# Autodesk Inventor assembly: Caja_Reductora
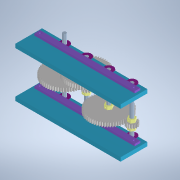
[picture p0: Inventor's stored thumbnail of the model, 180x180]
Saved by Autodesk Inventor 2022 (Build 260153000, 153)
## iProperties
Created: 2022-02-21
Part Number: Caja_Reductora
Document SubType Name: Assembly
Designer: katha
Author: katha
## Documents named in this file (11)
- C:\Users\katha\OneDrive\Escritorio\Mini_Proyecto_Diseno\Diseno_18012\Modelo_MPD\Caja_Reductora.iam
- C:\Users\katha\OneDrive\Escritorio\Mini_Proyecto_Diseno\Diseno_18012\Modelo_MPD\Engranajes_1_4.ipt
- C:\Users\katha\OneDrive\Escritorio\Mini_Proyecto_Diseno\Diseno_18012\Modelo_MPD\Engranajes_1_5.ipt
- C:\Users\katha\OneDrive\Escritorio\Mini_Proyecto_Diseno\Diseno_18012\Modelo_MPD\Eje1.ipt
- C:\Users\katha\OneDrive\Escritorio\Mini_Proyecto_Diseno\Diseno_18012\Modelo_MPD\Eje2.ipt
- C:\Users\katha\OneDrive\Escritorio\Mini_Proyecto_Diseno\Diseno_18012\Modelo_MPD\Hombro_Ejes.ipt
- C:\Users\katha\OneDrive\Escritorio\Mini_Proyecto_Diseno\Diseno_18012\Modelo_MPD\Rodamiento_Ejes.ipt
- C:\Users\katha\OneDrive\Escritorio\Mini_Proyecto_Diseno\Diseno_18012\Modelo_MPD\Carcasa_CajaR_Lateral1.ipt
- C:\Users\katha\OneDrive\Escritorio\Mini_Proyecto_Diseno\Diseno_18012\Modelo_MPD\Eje_Entrada.ipt
- C:\Users\katha\OneDrive\Escritorio\Mini_Proyecto_Diseno\Diseno_18012\Modelo_MPD\Eje_Salida.ipt
- C:\Users\katha\OneDrive\Escritorio\Mini_Proyecto_Diseno\Diseno_18012\Modelo_MPD\Carcasa_Tope.ipt
## Components (33 placed, 10 different names)
1. Engranajes_1_4:1 — Mate:2, Mate:3, Mate:35, Mate:36, Mate:43, Mate:44, Mate:63, Mate:64
2. Engranajes_1_5:1 — Mate:8, Mate:9, Mate:41, Mate:42, Mate:45, Mate:46, Mate:70, Mate:71
3. Engranajes_1_5:2 — Mate:1, Mate:4, Mate:5, Mate:6, Mate:7, Mate:37, Mate:38, Mate:39, Mate:40
4. Eje1:1 — Mate:1, Mate:2, Mate:3, Mate:4, Mate:5, Mate:10, Mate:11, Mate:12, Mate:13, Mate:14, Mate:15, Mate:16, Mate:17, Flush:1, Flush:2, Mate:27, Mate:28, Flush:4, Mate:31, Mate:32, Flush:6, Flush:7, Flush:10, Flush:11
5. Eje2:1 — Mate:6, Mate:7, Mate:8, Mate:9, Mate:18, Mate:19, Mate:20, Mate:21, Mate:22, Mate:23, Mate:24, Mate:25, Mate:26, Flush:1, Flush:3, Mate:29, Mate:30, Flush:5, Mate:33, Mate:34, Flush:8, Flush:9, Flush:11, Flush:12
6. Hombro_Ejes:1 — Mate:10, Mate:11, Flush:7, Mate:37
7. Hombro_Ejes:2 — Mate:12, Mate:13, Mate:38
8. Hombro_Ejes:3 — Mate:14, Mate:15, Mate:36
9. Hombro_Ejes:4 — Mate:16, Mate:17, Flush:6, Mate:35
10. Hombro_Ejes:5 — Mate:22, Mate:25, Mate:26, Mate:40
11. Hombro_Ejes:6 — Mate:23, Mate:24, Mate:39
12. Hombro_Ejes:7 — Mate:18, Mate:19, Flush:8, Mate:41
13. Hombro_Ejes:8 — Mate:20, Mate:21, Mate:42
14. Rodamiento_Ejes:1 — Flush:3, Mate:29, Mate:30, Flush:16
15. Rodamiento_Ejes:2 — Flush:2, Mate:27, Mate:28
16. Rodamiento_Ejes:3 — Flush:5, Mate:33, Mate:34
17. Rodamiento_Ejes:4 — Flush:4, Mate:31, Mate:32, Flush:13, Flush:19
18. Carcasa_CajaR_Lateral1:1 — Flush:9, Flush:17, Flush:18, Flush:20, Mate:56
19. Eje_Entrada:1 — Mate:43, Mate:44, Flush:10, Mate:47, Mate:48, Mate:52, Mate:53, Flush:15, Mate:59, Mate:60, Mate:61, Mate:62
20. Eje_Salida:1 — Mate:45, Mate:46, Flush:12, Mate:49, Mate:50, Mate:51, Flush:14, Mate:54, Mate:55, Mate:65, Mate:66, Mate:67, Mate:68, Mate:69
21. Rodamiento_Ejes:5 — Mate:47, Mate:48, Flush:13
22. Rodamiento_Ejes:6 — Mate:49, Mate:50, Mate:51, Flush:14
23. Rodamiento_Ejes:7 — Mate:52, Mate:53, Flush:15
24. Rodamiento_Ejes:8 — Mate:54, Mate:55, Flush:16
25. Carcasa_CajaR_Lateral1:2 — Flush:17, Flush:18, Flush:19, Mate:57, Mate:58
26. Carcasa_Tope:1 — Flush:20, Flush:21, Flush:22, Flush:23, Flush:24, Flush:25
27. Carcasa_Tope:2 — Flush:21, Flush:22, Mate:56
28. Carcasa_Tope:3 — Flush:23, Flush:24, Flush:26, Mate:57
29. Carcasa_Tope:4 — Flush:25, Flush:26, Mate:58
30. Hombro_Ejes:9 — Mate:59, Mate:60, Mate:64
31. Hombro_Ejes:10 — Mate:61, Mate:62, Mate:63
32. Hombro_Ejes:11 — Mate:65, Mate:68, Mate:69, Mate:70
33. Hombro_Ejes:12 — Mate:66, Mate:67, Mate:71
## Relationships (97: Mate 71, Flush 26)
- Mate:1 (0.3 mm): Engranajes_1_5:2 ↔ Eje1:1
- Mate:2 (0.3 mm): Engranajes_1_4:1 ↔ Eje1:1
- Mate:3 (0.3 mm): Engranajes_1_4:1 ↔ Eje1:1
- Mate:4 (0.3 mm): Engranajes_1_5:2 ↔ Eje1:1
- Mate:5 (0.3 mm): Engranajes_1_5:2 ↔ Eje1:1
- Mate:6 (0.3 mm): Engranajes_1_5:2 ↔ Eje2:1
- Mate:7 (0.3 mm): Engranajes_1_5:2 ↔ Eje2:1
- Mate:8 (0.3 mm): Engranajes_1_5:1 ↔ Eje2:1
- Mate:9 (0.3 mm): Engranajes_1_5:1 ↔ Eje2:1
- Mate:10 (0.3 mm): Eje1:1 ↔ Hombro_Ejes:1
- Mate:11 (0.3 mm): Eje1:1 ↔ Hombro_Ejes:1
- Mate:12 (0.3 mm): Eje1:1 ↔ Hombro_Ejes:2
- Mate:13 (0.3 mm): Eje1:1 ↔ Hombro_Ejes:2
- Mate:14 (0.3 mm): Eje1:1 ↔ Hombro_Ejes:3
- Mate:15 (0.3 mm): Eje1:1 ↔ Hombro_Ejes:3
- Mate:16 (0.3 mm): Eje1:1 ↔ Hombro_Ejes:4
- Mate:17 (0.3 mm): Eje1:1 ↔ Hombro_Ejes:4
- Mate:18 (0.3 mm): Eje2:1 ↔ Hombro_Ejes:7
- Mate:19 (0.3 mm): Eje2:1 ↔ Hombro_Ejes:7
- Mate:20 (0.3 mm): Eje2:1 ↔ Hombro_Ejes:8
- Mate:21 (0.3 mm): Eje2:1 ↔ Hombro_Ejes:8
- Mate:22 (0.3 mm): Eje2:1 ↔ Hombro_Ejes:5
- Mate:23 (0.3 mm): Eje2:1 ↔ Hombro_Ejes:6
- Mate:24 (0.3 mm): Eje2:1 ↔ Hombro_Ejes:6
- Mate:25 (0.3 mm): Eje2:1 ↔ Hombro_Ejes:5
- Mate:26 (0.3 mm): Eje2:1 ↔ Hombro_Ejes:5
- Flush:1: Eje1:1 ↔ Eje2:1
- Flush:2: Eje1:1 ↔ Rodamiento_Ejes:2
- Mate:27 (0.3 mm): Eje1:1 ↔ Rodamiento_Ejes:2
- Mate:28 (0.3 mm): Eje1:1 ↔ Rodamiento_Ejes:2
- Flush:3: Eje2:1 ↔ Rodamiento_Ejes:1
- Mate:29 (0.3 mm): Eje2:1 ↔ Rodamiento_Ejes:1
- Mate:30 (0.3 mm): Eje2:1 ↔ Rodamiento_Ejes:1
- Flush:4: Eje1:1 ↔ Rodamiento_Ejes:4
- Mate:31 (0.3 mm): Eje1:1 ↔ Rodamiento_Ejes:4
- Mate:32 (0.3 mm): Eje1:1 ↔ Rodamiento_Ejes:4
- Flush:5: Eje2:1 ↔ Rodamiento_Ejes:3
- Mate:33 (0.3 mm): Eje2:1 ↔ Rodamiento_Ejes:3
- Mate:34 (0.3 mm): Eje2:1 ↔ Rodamiento_Ejes:3
- Flush:6 (-15 mm): Eje1:1 ↔ Hombro_Ejes:4
- Mate:35 (0.1 mm): Engranajes_1_4:1 ↔ Hombro_Ejes:4
- Mate:36 (0.1 mm): Engranajes_1_4:1 ↔ Hombro_Ejes:3
- Flush:7 (15 mm): Eje1:1 ↔ Hombro_Ejes:1
- Mate:37 (0.1 mm): Engranajes_1_5:2 ↔ Hombro_Ejes:1
- Mate:38 (0.1 mm): Engranajes_1_5:2 ↔ Hombro_Ejes:2
- Mate:39 (0.1 mm): Engranajes_1_5:2 ↔ Hombro_Ejes:6
- Mate:40 (0.1 mm): Engranajes_1_5:2 ↔ Hombro_Ejes:5
- Flush:8 (28 mm): Eje2:1 ↔ Hombro_Ejes:7
- Mate:41 (0.1 mm): Engranajes_1_5:1 ↔ Hombro_Ejes:7
- Mate:42 (0.1 mm): Engranajes_1_5:1 ↔ Hombro_Ejes:8
- Flush:9: Eje2:1 ↔ Carcasa_CajaR_Lateral1:1
- Mate:43 (0.3 mm): Engranajes_1_4:1 ↔ Eje_Entrada:1
- Mate:44 (0.3 mm): Engranajes_1_4:1 ↔ Eje_Entrada:1
- Flush:10: Eje1:1 ↔ Eje_Entrada:1
- Flush:11: Eje1:1 ↔ Eje2:1
- Mate:45 (0.3 mm): Engranajes_1_5:1 ↔ Eje_Salida:1
- Mate:46 (0.3 mm): Engranajes_1_5:1 ↔ Eje_Salida:1
- Flush:12: Eje2:1 ↔ Eje_Salida:1
- Mate:47 (0.3 mm): Eje_Entrada:1 ↔ Rodamiento_Ejes:5
- Mate:48 (0.3 mm): Eje_Entrada:1 ↔ Rodamiento_Ejes:5
- Flush:13: Rodamiento_Ejes:4 ↔ Rodamiento_Ejes:5
- Mate:49 (0.3 mm): Eje_Salida:1 ↔ Rodamiento_Ejes:6
- Mate:50 (0.3 mm): Eje_Salida:1 ↔ Rodamiento_Ejes:6
- Mate:51 (0.3 mm): Eje_Salida:1 ↔ Rodamiento_Ejes:6
- Flush:14: Eje_Salida:1 ↔ Rodamiento_Ejes:6
- Mate:52 (0.3 mm): Eje_Entrada:1 ↔ Rodamiento_Ejes:7
- Mate:53 (0.3 mm): Eje_Entrada:1 ↔ Rodamiento_Ejes:7
- Flush:15: Eje_Entrada:1 ↔ Rodamiento_Ejes:7
- Mate:54 (0.3 mm): Eje_Salida:1 ↔ Rodamiento_Ejes:8
- Mate:55 (0.3 mm): Eje_Salida:1 ↔ Rodamiento_Ejes:8
- Flush:16: Rodamiento_Ejes:1 ↔ Rodamiento_Ejes:8
- Flush:17: Carcasa_CajaR_Lateral1:1 ↔ Carcasa_CajaR_Lateral1:2
- Flush:18: Carcasa_CajaR_Lateral1:1 ↔ Carcasa_CajaR_Lateral1:2
- Flush:19 (0.1 mm): Rodamiento_Ejes:4 ↔ Carcasa_CajaR_Lateral1:2
- Flush:20: Carcasa_CajaR_Lateral1:1 ↔ Carcasa_Tope:1
- Flush:21: Carcasa_Tope:1 ↔ Carcasa_Tope:2
- Flush:22: Carcasa_Tope:1 ↔ Carcasa_Tope:2
- Mate:56: Carcasa_CajaR_Lateral1:1 ↔ Carcasa_Tope:2
- Flush:23: Carcasa_Tope:1 ↔ Carcasa_Tope:3
- Flush:24: Carcasa_Tope:1 ↔ Carcasa_Tope:3
- Flush:25: Carcasa_Tope:1 ↔ Carcasa_Tope:4
- Flush:26: Carcasa_Tope:3 ↔ Carcasa_Tope:4
- Mate:57: Carcasa_CajaR_Lateral1:2 ↔ Carcasa_Tope:3
- Mate:58: Carcasa_CajaR_Lateral1:2 ↔ Carcasa_Tope:4
- Mate:59 (0.3 mm): Eje_Entrada:1 ↔ Hombro_Ejes:9
- Mate:60 (0.3 mm): Eje_Entrada:1 ↔ Hombro_Ejes:9
- Mate:61 (0.3 mm): Eje_Entrada:1 ↔ Hombro_Ejes:10
- Mate:62 (0.3 mm): Eje_Entrada:1 ↔ Hombro_Ejes:10
- Mate:63 (0.1 mm): Engranajes_1_4:1 ↔ Hombro_Ejes:10
- Mate:64 (0.1 mm): Engranajes_1_4:1 ↔ Hombro_Ejes:9
- Mate:65 (0.3 mm): Eje_Salida:1 ↔ Hombro_Ejes:11
- Mate:66 (0.3 mm): Eje_Salida:1 ↔ Hombro_Ejes:12
- Mate:67 (0.3 mm): Eje_Salida:1 ↔ Hombro_Ejes:12
- Mate:68 (0.3 mm): Eje_Salida:1 ↔ Hombro_Ejes:11
- Mate:69 (0.3 mm): Eje_Salida:1 ↔ Hombro_Ejes:11
- Mate:70 (0.1 mm): Engranajes_1_5:1 ↔ Hombro_Ejes:11
- Mate:71 (0.1 mm): Engranajes_1_5:1 ↔ Hombro_Ejes:12
